# Autodesk Inventor assembly: VersaPlanetary_v2_Two_Stage_100_1_with_BAG
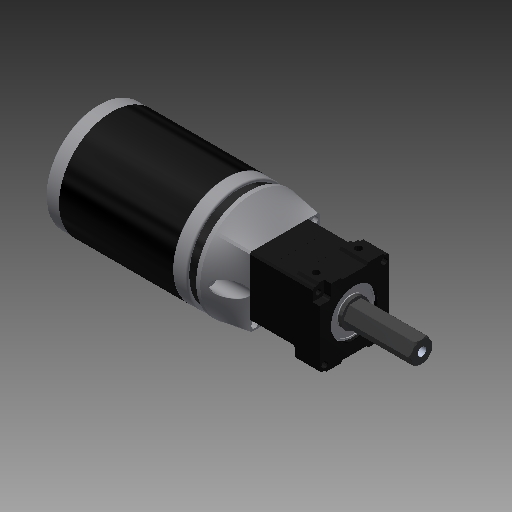
[picture p0: Inventor's stored thumbnail of the model, 512x512]
Saved by Autodesk Inventor 2017 (Build 210142000, 142)
## iProperties
Created: 2016-10-31
Part Number: VersaPlanetary_v2_Two_Stage_100_1_with_BAG
Description: STEP AP214
Document SubType Name: Assembly
Designer: S331461152
Sending System: SolidWorks 2016
Preprocessor: SwSTEP 2.0
Title: 217-4973_2stage_BAG.STEP
Revision Number: ANY
## Documents named in this file (14)
- \\ad.ocdsb.ca\studenthome\5\S346795925\Robotics\698590_FRC_Season_2017_18_c6a29b2db01e1b8a_1517863524\Robot Mostly Finalized V16\VersaPlanetary_v2_Two_Stage_100_1_with_BAG.iam
- \\ad.ocdsb.ca\studenthome\5\S346795925\Robotics\698590_FRC_Season_2017_18_c6a29b2db01e1b8a_1517863524\Robot Mostly Finalized V16\217-2625-026 Rev1.ipt
- \\ad.ocdsb.ca\studenthome\5\S346795925\Robotics\698590_FRC_Season_2017_18_c6a29b2db01e1b8a_1517863524\Robot Mostly Finalized V16\217-2742-001 Rev4.ipt
- \\ad.ocdsb.ca\studenthome\5\S346795925\Robotics\698590_FRC_Season_2017_18_c6a29b2db01e1b8a_1517863524\Robot Mostly Finalized V16\217-2625-017 Rev1_9714K61.ipt
- \\ad.ocdsb.ca\studenthome\5\S346795925\Robotics\698590_FRC_Season_2017_18_c6a29b2db01e1b8a_1517863524\Robot Mostly Finalized V16\217-2625-003 Rev1.ipt
- \\ad.ocdsb.ca\studenthome\5\S346795925\Robotics\698590_FRC_Season_2017_18_c6a29b2db01e1b8a_1517863524\Robot Mostly Finalized V16\217-2625-018 Rev1_98541A410.ipt
- \\ad.ocdsb.ca\studenthome\5\S346795925\Robotics\698590_FRC_Season_2017_18_c6a29b2db01e1b8a_1517863524\Robot Mostly Finalized V16\217-2820 Rev1_Public.iam
- \\ad.ocdsb.ca\studenthome\5\S346795925\Robotics\698590_FRC_Season_2017_18_c6a29b2db01e1b8a_1517863524\Robot Mostly Finalized V16\217-2816-001 Rev1.ipt
- \\ad.ocdsb.ca\studenthome\5\S346795925\Robotics\698590_FRC_Season_2017_18_c6a29b2db01e1b8a_1517863524\Robot Mostly Finalized V16\217-4649-001 Rev1.ipt
- \\ad.ocdsb.ca\studenthome\5\S346795925\Robotics\698590_FRC_Season_2017_18_c6a29b2db01e1b8a_1517863524\Robot Mostly Finalized V16\217-4649-007 Rev1_94105A824.ipt
- \\ad.ocdsb.ca\studenthome\5\S346795925\Robotics\698590_FRC_Season_2017_18_c6a29b2db01e1b8a_1517863524\Robot Mostly Finalized V16\217-2625-011 Rev1.ipt
- \\ad.ocdsb.ca\studenthome\5\S346795925\Robotics\698590_FRC_Season_2017_18_c6a29b2db01e1b8a_1517863524\Robot Mostly Finalized V16\Mini_CIM_Motor_217-3371.ipt
- \\ad.ocdsb.ca\studenthome\5\S346795925\Robotics\698590_FRC_Season_2017_18_c6a29b2db01e1b8a_1517863524\Robot Mostly Finalized V16\VersaPlanetary_CIM_Adapter_217-4018.ipt
- \\ad.ocdsb.ca\studenthome\5\S346795925\Robotics\698590_FRC_Season_2017_18_c6a29b2db01e1b8a_1517863524\Robot Mostly Finalized V16\am-3314a+CIMcoder+V2.iam
## Components (16 placed, 16 different names)
1. 217-2625-026 Rev1_1
2. 217-2742-001 Rev4_2
3. 217-2742-001 Rev4_3
4. 217-2625-017 Rev1_9714K61_4
5. 217-2625-003 Rev1_5
6. 217-2625-018 Rev1_98541A410_6
7. 217-2820 Rev1_Public_16 [sub-assembly]
8. 217-2816-001 Rev1_17
9. 217-2820 Rev1_Public_18 [sub-assembly]
10. 217-2816-001 Rev1_19 — Mate:5, Mate:6
11. 217-4649-001 Rev1_20
12. 217-4649-007 Rev1_94105A824_21
13. 217-2625-011 Rev1_22
14. Mini_CIM_Motor_217-3371:1 — Mate:1, Mate:7, Mate:8, Mate:9
15. VersaPlanetary_CIM_Adapter_217-4018:1 — Mate:1, Mate:5, Mate:6, Mate:7, Mate:10
16. am-3314a+CIMcoder+V2:1 [sub-assembly] — Mate:8, Mate:9, Mate:10
## Relationships (7: Mate 7)
- Mate:1: Mini_CIM_Motor_217-3371:1 ↔ VersaPlanetary_CIM_Adapter_217-4018:1
- Mate:5: 217-2816-001 Rev1_19 ↔ VersaPlanetary_CIM_Adapter_217-4018:1
- Mate:6: 217-2816-001 Rev1_19 ↔ VersaPlanetary_CIM_Adapter_217-4018:1
- Mate:7: Mini_CIM_Motor_217-3371:1 ↔ VersaPlanetary_CIM_Adapter_217-4018:1
- Mate:8: Mini_CIM_Motor_217-3371:1 ↔ am-3314a+CIMcoder+V2:1
- Mate:9: Mini_CIM_Motor_217-3371:1 ↔ am-3314a+CIMcoder+V2:1
- Mate:10: VersaPlanetary_CIM_Adapter_217-4018:1 ↔ am-3314a+CIMcoder+V2:1
